# Autodesk Inventor assembly: Robot
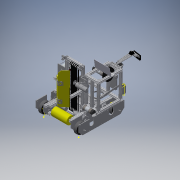
[picture p0: Inventor's stored thumbnail of the model, 180x180]
Saved by Autodesk Inventor 2016 (Build 200138000, 138)
## iProperties
Created: 2016-10-08
Part Number: Robot
Document SubType Name: Assembly
Designer: RoboticsUser
Author: RoboticsUser
## Documents named in this file (26)
- C:\Robotics\CAD\2016-17_CAD\Robot.iam
- C:\Robotics\CAD\2016-17_CAD\WheelAssemblyWFrame.iam
- C:\Robotics\CAD\COTSParts\Bosch Extrusion\Bosch 20x20 9 in.ipt
- C:\Robotics\CAD\COTSParts\Bosch Extrusion\Gusset 20x20 w screws.ipt
- C:\Robotics\CAD\COTSParts\Bosch Extrusion\Bosch 20x20 9 in - Copy.ipt
- C:\Robotics\CAD\COTSParts\Bosch Extrusion\Rexroth-6mmT-Nutm4.ipt
- C:\Robotics\CAD\COTSParts\Bosch Extrusion\Rexroth-GussetwFastenersm4x8.ipt
- C:\Robotics\CAD\COTSParts\Bosch Extrusion\Bosch 20x20 8.937in.ipt
- C:\Robotics\CAD\2016-17_CAD\ParticleLauncher2.0.iam
- C:\Robotics\CAD\2016-17_CAD\BBP.iam
- C:\Robotics\CAD\2016-17_CAD\ElectronicsPlate2.ipt
- C:\Robotics\CAD\2016-17_CAD\Deflecter.ipt
- C:\Robotics\CAD\COTSParts\Actobotics\585 parts\585424.ipt
- C:\Robotics\CAD\2016-17_CAD\14inLift - Copy.iam
- C:\Robotics\CAD\COTSParts\Bosch Extrusion\Bosch 20x20 4 14in.ipt
- C:\Robotics\CAD\2016-17_CAD\Backstop.iam
- C:\Robotics\CAD\COTSParts\Bosch Extrusion\Bosch 20x20 9 in actual2.ipt
- C:\Robotics\CAD\2016-17_CAD\CollectorPrototype.iam
- C:\Robotics\CAD\COTSParts\Actobotics\585 parts\585494.ipt
- C:\Robotics\CAD\COTSParts\Motors\Andymark 2964  NeveRest 40 Motor.ipt
- C:\Robotics\CAD\COTSParts\Actobotics\555 parts\555116.ipt
- C:\Robotics\CAD\2016-17_CAD\Motorstandoff1a1.2.ipt
- C:\Robotics\CAD\COTSParts\Actobotics\615 parts\615102.ipt
- C:\Robotics\CAD\2016-17_CAD\ModuleAssembly.iam
- C:\Robotics\CAD\COTSParts\ModernRobotics\MRI45-2203_Motor_Controller.ipt
- C:\Robotics\CAD\2016-17_CAD\Phone.ipt
## Components (50 placed, 25 different names)
1. WheelAssemblyWFrame:1 [sub-assembly] — Mate:1, Insert:4, Insert:5, Insert:6, Flush:29, Flush:37, Flush:42, Flush:114, Mate:181
2. WheelAssemblyWFrame:2 [sub-assembly] — Mate:8, Insert:1, Insert:2, Insert:3, Flush:30, Mate:57, Mate:58, Mate:77, Mate:192, Mate:194, Flush:122, Flush:123, Mate:198, Flush:124, Mate:201, Flush:125, Mate:203, Flush:126
3. Bosch 20x20 9 in:1 — Flush:37, Mate:56, Mate:58, Flush:42, Mate:77, Mate:180
4. Gusset 20x20 w screws:2 — Mate:1
5. Gusset 20x20 w screws:3 — Mate:8
6. Bosch 20x20 9 in - Copy:1 — Mate:33, Flush:25, Flush:28, Flush:30, Mate:44, Flush:34, Mate:175, Mate:183, Flush:115
7. Rexroth-6mmT-Nutm4:1 — Insert:1
8. Rexroth-6mmT-Nutm4:2 — Insert:3, Mate:33, Flush:25
9. Rexroth-6mmT-Nutm4:3 — Insert:2
10. Bosch 20x20 9 in - Copy:2 — Mate:15, Flush:11, Mate:39, Flush:29, Flush:32, Mate:48, Flush:33, Flush:116
11. Rexroth-6mmT-Nutm4:4 — Insert:4
12. Rexroth-6mmT-Nutm4:5 — Insert:5
13. Rexroth-6mmT-Nutm4:6 — Insert:6, Mate:15, Flush:11
14. Bosch 20x20 9 in:4 — Mate:39, Flush:28, Flush:32, Mate:45, Mate:46, Mate:47, Mate:49, Flush:33, Flush:34, Flush:111
15. Gusset 20x20 w screws:7 — Mate:47, Mate:48, Mate:49
16. Gusset 20x20 w screws:8 — Mate:44, Mate:45, Mate:46
17. Rexroth-GussetwFastenersm4x8:4 — Mate:56, Mate:57
18. Bosch 20x20 8.937in:4 — Mate:93, Flush:62, Flush:92, Flush:103, Flush:104, Mate:160
19. ParticleLauncher2.0:1 [sub-assembly] — Flush:103, Flush:104, Mate:160, Mate:163, Mate:164, Mate:165, Mate:166, Mate:168, Mate:169, Mate:170, Mate:171, Mate:174, Flush:113, Flush:114, Mate:180, Mate:181, Mate:206, Flush:127, Mate:207, Mate:208, Mate:209
20. Gusset 20x20 w screws:18 — Mate:93, Flush:62, Flush:92
21. BBP:1 [sub-assembly] — Mate:206, Flush:127, Mate:207
22. ElectronicsPlate2:1 — Mate:175, Flush:111
23. Deflecter:2 — Mate:174, Mate:177, Flush:112, Mate:179
24. 585424:2 — Insert:7, Insert:8, Flush:112, Mate:179, Flush:113
25. Rexroth-6mmT-Nutm4:7 — Mate:165, Mate:166, Insert:9
26. Rexroth-6mmT-Nutm4:8 — Mate:163, Mate:164, Insert:10
27. Rexroth-6mmT-Nutm4:10 — Mate:168, Mate:169, Insert:8
28. Rexroth-6mmT-Nutm4:11 — Mate:170, Mate:171, Insert:7
29. 585424:3 — Insert:9, Insert:10, Mate:177
30. 14inLift - Copy:1 [sub-assembly] — Mate:183, Flush:115, Flush:116, Mate:184, Flush:117, Mate:187, Mate:188, Flush:118, Mate:193, Flush:119, Flush:120, Flush:121, Mate:195, Mate:196, Mate:197, Insert:18, Mate:199
31. Bosch 20x20 4 14in:1 — Mate:184, Flush:117, Mate:185
32. Backstop:1 [sub-assembly] — Mate:185, Mate:190, Mate:191
33. Bosch 20x20 4 14in:2 — Mate:188, Flush:118, Mate:191, Flush:121
34. Bosch 20x20 4 14in:3 — Mate:187, Mate:190, Flush:120
35. Bosch 20x20 9 in actual2:1 — Mate:192, Mate:193, Flush:119
36. CollectorPrototype:1 [sub-assembly] — Mate:194, Flush:122, Flush:123
37. 585494:1 — Insert:11, Insert:12, Insert:13, Insert:14
38. Andymark 2964  NeveRest 40 Motor:1 — Insert:15, Insert:19
39. 555116:1 — Insert:15, Insert:16, Insert:17
40. Motorstandoff1a1.2:1 — Insert:12, Insert:17
41. Motorstandoff1a1.2:2 — Insert:11, Insert:16
42. Rexroth-6mmT-Nutm4:12 — Insert:13, Mate:195, Mate:196
43. Rexroth-6mmT-Nutm4:13 — Insert:14, Mate:197
44. 615102:1 — Insert:18
45. 615102:2 — Insert:19
46. ModuleAssembly:1 [sub-assembly] — Mate:198, Mate:199, Flush:124, Mate:200, Mate:202, Mate:204, Mate:205
47. Gusset 20x20 w screws:23 — Mate:200, Mate:201, Flush:125
48. Gusset 20x20 w screws:24 — Mate:202, Mate:203, Flush:126
49. MRI45-2203_Motor_Controller:2 — Mate:204, Mate:205
50. Phone:1 — Mate:208, Mate:209
## Relationships (106: Mate 56, Flush 31, Insert 19)
- Mate:1: WheelAssemblyWFrame:1 ↔ Gusset 20x20 w screws:2
- Mate:8: WheelAssemblyWFrame:2 ↔ Gusset 20x20 w screws:3
- Insert:1: WheelAssemblyWFrame:2 ↔ Rexroth-6mmT-Nutm4:1
- Insert:2: WheelAssemblyWFrame:2 ↔ Rexroth-6mmT-Nutm4:3
- Insert:3: WheelAssemblyWFrame:2 ↔ Rexroth-6mmT-Nutm4:2
- Insert:4: WheelAssemblyWFrame:1 ↔ Rexroth-6mmT-Nutm4:4
- Insert:5: WheelAssemblyWFrame:1 ↔ Rexroth-6mmT-Nutm4:5
- Insert:6: WheelAssemblyWFrame:1 ↔ Rexroth-6mmT-Nutm4:6
- Mate:15: Bosch 20x20 9 in - Copy:2 ↔ Rexroth-6mmT-Nutm4:6
- Flush:11 (64.77 mm): Bosch 20x20 9 in - Copy:2 ↔ Rexroth-6mmT-Nutm4:6
- Mate:33: Bosch 20x20 9 in - Copy:1 ↔ Rexroth-6mmT-Nutm4:2
- Flush:25 (64.77 mm): Bosch 20x20 9 in - Copy:1 ↔ Rexroth-6mmT-Nutm4:2
- Mate:39: Bosch 20x20 9 in - Copy:2 ↔ Bosch 20x20 9 in:4
- Flush:28: Bosch 20x20 9 in - Copy:1 ↔ Bosch 20x20 9 in:4
- Flush:29 (1.6256 mm): WheelAssemblyWFrame:1 ↔ Bosch 20x20 9 in - Copy:2
- Flush:30 (1.6256 mm): WheelAssemblyWFrame:2 ↔ Bosch 20x20 9 in - Copy:1
- Flush:32: Bosch 20x20 9 in - Copy:2 ↔ Bosch 20x20 9 in:4
- Mate:44: Bosch 20x20 9 in - Copy:1 ↔ Gusset 20x20 w screws:8
- Mate:45: Bosch 20x20 9 in:4 ↔ Gusset 20x20 w screws:8
- Mate:46: Bosch 20x20 9 in:4 ↔ Gusset 20x20 w screws:8
- Mate:47: Bosch 20x20 9 in:4 ↔ Gusset 20x20 w screws:7
- Mate:48: Bosch 20x20 9 in - Copy:2 ↔ Gusset 20x20 w screws:7
- Mate:49: Bosch 20x20 9 in:4 ↔ Gusset 20x20 w screws:7
- Flush:33: Bosch 20x20 9 in - Copy:2 ↔ Bosch 20x20 9 in:4
- Flush:34: Bosch 20x20 9 in - Copy:1 ↔ Bosch 20x20 9 in:4
- Flush:37: WheelAssemblyWFrame:1 ↔ Bosch 20x20 9 in:1
- Mate:56: Bosch 20x20 9 in:1 ↔ Rexroth-GussetwFastenersm4x8:4
- Mate:57: WheelAssemblyWFrame:2 ↔ Rexroth-GussetwFastenersm4x8:4
- Mate:58: WheelAssemblyWFrame:2 ↔ Bosch 20x20 9 in:1
- Flush:42: WheelAssemblyWFrame:1 ↔ Bosch 20x20 9 in:1
- Mate:77: WheelAssemblyWFrame:2 ↔ Bosch 20x20 9 in:1
- Mate:93: Bosch 20x20 8.937in:4 ↔ Gusset 20x20 w screws:18
- Flush:62: Bosch 20x20 8.937in:4 ↔ Gusset 20x20 w screws:18
- Flush:92: Bosch 20x20 8.937in:4 ↔ Gusset 20x20 w screws:18
- Flush:103: Bosch 20x20 8.937in:4 ↔ ParticleLauncher2.0:1
- Flush:104: Bosch 20x20 8.937in:4 ↔ ParticleLauncher2.0:1
- Mate:160: Bosch 20x20 8.937in:4 ↔ ParticleLauncher2.0:1
- Mate:163: ParticleLauncher2.0:1 ↔ Rexroth-6mmT-Nutm4:8
- Mate:164: ParticleLauncher2.0:1 ↔ Rexroth-6mmT-Nutm4:8
- Mate:165: ParticleLauncher2.0:1 ↔ Rexroth-6mmT-Nutm4:7
- Mate:166: ParticleLauncher2.0:1 ↔ Rexroth-6mmT-Nutm4:7
- Mate:168: ParticleLauncher2.0:1 ↔ Rexroth-6mmT-Nutm4:10
- Mate:169: ParticleLauncher2.0:1 ↔ Rexroth-6mmT-Nutm4:10
- Mate:170: ParticleLauncher2.0:1 ↔ Rexroth-6mmT-Nutm4:11
- Mate:171: ParticleLauncher2.0:1 ↔ Rexroth-6mmT-Nutm4:11
- Mate:174: ParticleLauncher2.0:1 ↔ Deflecter:2
- Mate:175: Bosch 20x20 9 in - Copy:1 ↔ ElectronicsPlate2:1
- Flush:111 (7.3914 mm): Bosch 20x20 9 in:4 ↔ ElectronicsPlate2:1
- Insert:7: 585424:2 ↔ Rexroth-6mmT-Nutm4:11
- Insert:8: 585424:2 ↔ Rexroth-6mmT-Nutm4:10
- Insert:9: Rexroth-6mmT-Nutm4:7 ↔ 585424:3
- Insert:10: Rexroth-6mmT-Nutm4:8 ↔ 585424:3
- Mate:177: Deflecter:2 ↔ 585424:3
- Flush:112 (2.54 mm): Deflecter:2 ↔ 585424:2
- Mate:179: Deflecter:2 ↔ 585424:2
- Flush:113 (-88.9 mm): ParticleLauncher2.0:1 ↔ 585424:2
- Flush:114: WheelAssemblyWFrame:1 ↔ ParticleLauncher2.0:1
- Mate:180: Bosch 20x20 9 in:1 ↔ ParticleLauncher2.0:1
- Mate:181: WheelAssemblyWFrame:1 ↔ ParticleLauncher2.0:1
- Mate:183: Bosch 20x20 9 in - Copy:1 ↔ 14inLift - Copy:1
- Flush:115: Bosch 20x20 9 in - Copy:1 ↔ 14inLift - Copy:1
- Flush:116 (114.3 mm): Bosch 20x20 9 in - Copy:2 ↔ 14inLift - Copy:1
- Mate:184: 14inLift - Copy:1 ↔ Bosch 20x20 4 14in:1
- Flush:117: 14inLift - Copy:1 ↔ Bosch 20x20 4 14in:1
- Mate:185: Bosch 20x20 4 14in:1 ↔ Backstop:1
- Mate:187: 14inLift - Copy:1 ↔ Bosch 20x20 4 14in:3
- Mate:188: 14inLift - Copy:1 ↔ Bosch 20x20 4 14in:2
- Flush:118 (76.2 mm): 14inLift - Copy:1 ↔ Bosch 20x20 4 14in:2
- Mate:190: Backstop:1 ↔ Bosch 20x20 4 14in:3
- Mate:191: Backstop:1 ↔ Bosch 20x20 4 14in:2
- Mate:192: WheelAssemblyWFrame:2 ↔ Bosch 20x20 9 in actual2:1
- Mate:193: 14inLift - Copy:1 ↔ Bosch 20x20 9 in actual2:1
- Flush:119: 14inLift - Copy:1 ↔ Bosch 20x20 9 in actual2:1
- Flush:120: 14inLift - Copy:1 ↔ Bosch 20x20 4 14in:3
- Flush:121: 14inLift - Copy:1 ↔ Bosch 20x20 4 14in:2
- Mate:194: WheelAssemblyWFrame:2 ↔ CollectorPrototype:1
- Flush:122: WheelAssemblyWFrame:2 ↔ CollectorPrototype:1
- Flush:123 (25.4 mm): WheelAssemblyWFrame:2 ↔ CollectorPrototype:1
- Insert:11: 585494:1 ↔ Motorstandoff1a1.2:2
- Insert:12: 585494:1 ↔ Motorstandoff1a1.2:1
- Insert:13: 585494:1 ↔ Rexroth-6mmT-Nutm4:12
- Insert:14: 585494:1 ↔ Rexroth-6mmT-Nutm4:13
- Insert:15: Andymark 2964  NeveRest 40 Motor:1 ↔ 555116:1
- Insert:16: 555116:1 ↔ Motorstandoff1a1.2:2
- Insert:17: 555116:1 ↔ Motorstandoff1a1.2:1
- Mate:195: 14inLift - Copy:1 ↔ Rexroth-6mmT-Nutm4:12
- Mate:196: 14inLift - Copy:1 ↔ Rexroth-6mmT-Nutm4:12
- Mate:197: 14inLift - Copy:1 ↔ Rexroth-6mmT-Nutm4:13
- Insert:18 (7.62 mm): 14inLift - Copy:1 ↔ 615102:1
- Insert:19 (2.54 mm): Andymark 2964  NeveRest 40 Motor:1 ↔ 615102:2
- Mate:198: WheelAssemblyWFrame:2 ↔ ModuleAssembly:1
- Mate:199: 14inLift - Copy:1 ↔ ModuleAssembly:1
- Flush:124: WheelAssemblyWFrame:2 ↔ ModuleAssembly:1
- Mate:200: ModuleAssembly:1 ↔ Gusset 20x20 w screws:23
- Mate:201: WheelAssemblyWFrame:2 ↔ Gusset 20x20 w screws:23
- Flush:125: WheelAssemblyWFrame:2 ↔ Gusset 20x20 w screws:23
- Mate:202: ModuleAssembly:1 ↔ Gusset 20x20 w screws:24
- Mate:203: WheelAssemblyWFrame:2 ↔ Gusset 20x20 w screws:24
- Flush:126: WheelAssemblyWFrame:2 ↔ Gusset 20x20 w screws:24
- Mate:204: ModuleAssembly:1 ↔ MRI45-2203_Motor_Controller:2
- Mate:205: ModuleAssembly:1 ↔ MRI45-2203_Motor_Controller:2
- Mate:206: ParticleLauncher2.0:1 ↔ BBP:1
- Flush:127: ParticleLauncher2.0:1 ↔ BBP:1
- Mate:207: ParticleLauncher2.0:1 ↔ BBP:1
- Mate:208: ParticleLauncher2.0:1 ↔ Phone:1
- Mate:209: ParticleLauncher2.0:1 ↔ Phone:1
